# Autodesk Inventor assembly: PasekZNaciagiem
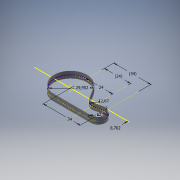
[picture p0: Inventor's stored thumbnail of the model, 180x180]
Saved by Autodesk Inventor 2019 (Build 230136000, 136)
## iProperties
Created: 2020-08-19
Part Number: PasekZNaciagiem
Document SubType Name: Assembly
Designer: estee
Author: estee
## Documents named in this file (4)
- C:\Users\estee\OneDrive\Pulpit\estere\1\MUM\projejt\PasekZNaciagiem.iam
- C:\Users\estee\OneDrive\Pulpit\estere\1\MUM\projejt\PasekZebaty — kopia.ipt
- C:\Users\estee\OneDrive\Pulpit\estere\1\MUM\projejt\zab.ipt
- C:\Users\estee\OneDrive\Pulpit\estere\1\MUM\projejt\PasekZebaty.ipt
## Components (3 placed, 3 different names)
1. PasekZebaty — kopia:1 — Mate:1, Angle:1, Mate:3, Mate:5, Flush:1
2. zab:1 — Mate:1, Mate:2, Angle:2, Mate:6
3. PasekZebaty:1 — Mate:4, Mate:5, Flush:1
## Relationships (9: Mate 6, Angle 2, Flush 1)
- Mate:1: PasekZebaty — kopia:1 ↔ zab:1
- Mate:2: zab:1
- Angle:1 (0 deg): PasekZebaty — kopia:1
- Mate:3: PasekZebaty — kopia:1
- Angle:2 (0 deg): zab:1
- Mate:4: PasekZebaty:1
- Mate:5: PasekZebaty — kopia:1 ↔ PasekZebaty:1
- Flush:1: PasekZebaty — kopia:1 ↔ PasekZebaty:1
- Mate:6: zab:1
